# Autodesk Inventor assembly: detectorArray
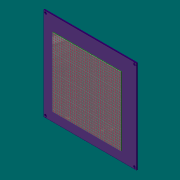
[picture p0: Inventor's stored thumbnail of the model, 180x180]
Saved by Autodesk Inventor 2016 SP2 (Build 200236200, 236)
## iProperties
Created: 2016-04-02
Part Number: detectorArray
Document SubType Name: Assembly
Designer: sawai
Author: sawai
## Documents named in this file (3)
- C:\Users\Sawaiz\oneDrive\projects\modularRICH\detector\detectorArray.iam
- C:\Users\Sawaiz\oneDrive\projects\modularRICH\dependency\13361-30xxAE-08\13361-30xxAE-08.iam
- C:\Users\Sawaiz\oneDrive\projects\modularRICH\dependency\modularRICHBackplane\cad\backplane.iam
## Components (17 placed, 2 different names)
1. backplane:1 [sub-assembly] — Mate:1
2. 13361-30xxAE-08:1 [sub-assembly]
3. 13361-30xxAE-08:2 [sub-assembly]
4. 13361-30xxAE-08:3 [sub-assembly]
5. 13361-30xxAE-08:4 [sub-assembly] — Mate:1
6. 13361-30xxAE-08:5 [sub-assembly]
7. 13361-30xxAE-08:6 [sub-assembly]
8. 13361-30xxAE-08:7 [sub-assembly]
9. 13361-30xxAE-08:8 [sub-assembly]
10. 13361-30xxAE-08:9 [sub-assembly]
11. 13361-30xxAE-08:10 [sub-assembly]
12. 13361-30xxAE-08:11 [sub-assembly]
13. 13361-30xxAE-08:12 [sub-assembly]
14. 13361-30xxAE-08:13 [sub-assembly]
15. 13361-30xxAE-08:14 [sub-assembly]
16. 13361-30xxAE-08:15 [sub-assembly]
17. 13361-30xxAE-08:16 [sub-assembly]
## Component patterns: (16 elements, first: 13361-30xxAE-08:1)
## Relationships (1: Mate 1)
- Mate:1: backplane:1 ↔ 13361-30xxAE-08:4
